# Autodesk Inventor assembly: FrameV2
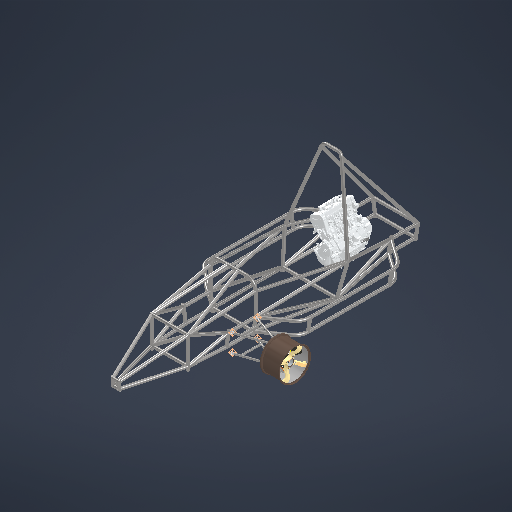
[picture p0: Inventor's stored thumbnail of the model, 512x512]
Saved by Autodesk Inventor 2026.2 (Build 302298010, 298A)
## iProperties
Created: 2026-06-05
Part Number: FrameV2
Document SubType Name: Assembly
Designer: tasle
_SolveAssemblyDoc: Frame Generator Solve Assembly
_Version: 25.0.0
Author: tasle
## Documents named in this file (6)
- C:\Users\tasle\Documents\PersonalProjects\FSAE\GOGO_FSAE_CAD\FrameV2.iam
- C:\Users\tasle\Documents\PersonalProjects\FSAE\GOGO_FSAE_CAD\PrelimFrame.ipt
- C:\Users\tasle\Documents\PersonalProjects\FSAE\GOGO_FSAE_CAD\FrameV2\Frame\Frame 1780692296746.iam
- C:\Users\tasle\Documents\PersonalProjects\FSAE\GOGO_FSAE_CAD\honda-cbr600-f4i-engine-1.snapshot.3\Honda CBR600 F4i\Honda CBR600 F4i\Honda CBR600 F4i.ipt
- C:\Users\tasle\Documents\PersonalProjects\FSAE\GOGO_FSAE_CAD\Suspension\Upright Assembly\Front Left Wheel Hub Assemby.iam
- C:\Users\tasle\Documents\PersonalProjects\FSAE\GOGO_FSAE_CAD\Suspension\Suspension Parts\Front Upper Arm\Front_Upper_Arm_Assembly.iam
## Components (6 placed, 5 different names)
1. PrelimFrame:1
2. Frame 1780692296746:1 [sub-assembly]
3. Honda CBR600 F4i:1
4. Front Left Wheel Hub Assemby:1 [sub-assembly] — Rotational:1, Rotational:2
5. Front_Upper_Arm_Assembly:1 [sub-assembly] — Rotational:1
6. Front_Upper_Arm_Assembly:2 [sub-assembly] — Rotational:2
## Relationships (2: RevoluteJoint 2)
- Rotational:1 [RevoluteJoint]: Front Left Wheel Hub Assemby:1 ↔ Front_Upper_Arm_Assembly:1
- Rotational:2 [RevoluteJoint]: Front Left Wheel Hub Assemby:1 ↔ Front_Upper_Arm_Assembly:2
